# Autodesk Inventor assembly: Assembly1
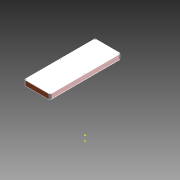
[picture p0: Inventor's stored thumbnail of the model, 180x180]
Saved by Autodesk Inventor 2015 (Build 190159000, 159)
## iProperties
Created: 2014-07-25
Part Number: Assembly1
Document SubType Name: Assembly
Designer: Michael
Author: Michael
## Documents named in this file (4)
- C:\Users\Michael\Dropbox\schwa42 (1)\case\3D\Assembly1.iam
- C:\Users\Michael\Dropbox\schwa42 (1)\case\3D\Base.ipt
- C:\Users\Michael\Dropbox\schwa42 (1)\case\3D\Mid.ipt
- C:\Users\Michael\Dropbox\schwa42 (1)\case\3D\Spacer.ipt
## Components (7 placed, 3 different names)
1. Base:1 — Flush:1, Flush:2, Mate:1, Mate:4, Mate:5, Mate:7, Mate:8
2. Base:2 — Flush:3, Flush:4, Mate:2, Mate:3, Mate:6
3. Mid:1 — Flush:1, Flush:2, Mate:1, Flush:3, Flush:4, Mate:2, Tangent:1, Tangent:2
4. Spacer:1 — Tangent:1, Mate:3
5. Spacer:2 — Tangent:2, Mate:4
6. Spacer:3 — Mate:5, Mate:6
7. Spacer:4 — Mate:7, Mate:8
## Relationships (14: Mate 8, Flush 4, Tangent 2)
- Flush:1: Base:1 ↔ Mid:1
- Flush:2: Base:1 ↔ Mid:1
- Mate:1: Base:1 ↔ Mid:1
- Flush:3: Base:2 ↔ Mid:1
- Flush:4: Base:2 ↔ Mid:1
- Mate:2: Base:2 ↔ Mid:1
- Tangent:1: Mid:1 ↔ Spacer:1
- Mate:3: Base:2 ↔ Spacer:1
- Tangent:2: Mid:1 ↔ Spacer:2
- Mate:4: Base:1 ↔ Spacer:2
- Mate:5: Base:1 ↔ Spacer:3
- Mate:6: Base:2 ↔ Spacer:3
- Mate:7: Base:1 ↔ Spacer:4
- Mate:8: Base:1 ↔ Spacer:4
